# Autodesk Inventor assembly: GarageAndBracket
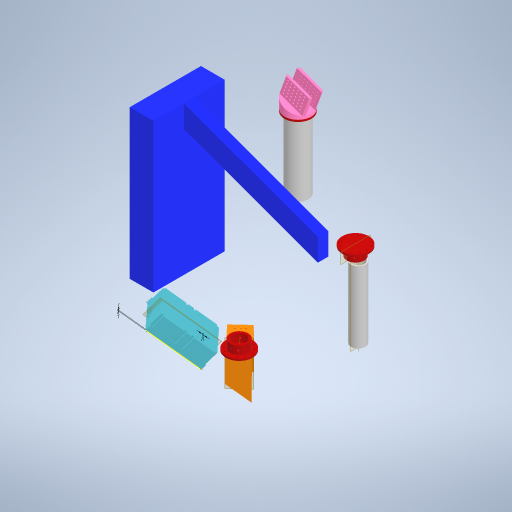
[picture p0: Inventor's stored thumbnail of the model, 512x512]
Saved by Autodesk Inventor 2023 (Build 270158030, 158C)
## iProperties
Created: 2021-11-26
Part Number: GarageAndBracket
Document SubType Name: Assembly
Designer: robst
Author: robst
## Documents named in this file (9)
- C:\git\CAD-Development\robSteele\ShapeWays\GlobalMeteorNetwork\GarageAndBracket.iam
- C:\git\CAD-Development\robSteele\ShapeWays\GlobalMeteorNetwork\GarageSegment.ipt
- C:\git\CAD-Development\robSteele\ShapeWays\GlobalMeteorNetwork\pvcBracketUpperPortionV02.ipt
- C:\git\CAD-Development\robSteele\ShapeWays\GlobalMeteorNetwork\topAttachementForPvcPipe.ipt
- C:\git\CAD-Development\robSteele\ShapeWays\GlobalMeteorNetwork\bracketForGarageLowerHalf.ipt
- C:\git\CAD-Development\robSteele\ShapeWays\GlobalMeteorNetwork\caseUpperPortion.ipt
- C:\git\CAD-Development\robSteele\ShapeWays\GlobalMeteorNetwork\3inchPvcPipe.ipt
- C:\git\CAD-Development\robSteele\ShapeWays\GlobalMeteorNetwork\2inchPvcForBracket.ipt
- C:\git\CAD-Development\robSteele\ShapeWays\GlobalMeteorNetwork\topAttachementFor2InchPvcPipe.ipt
## Components (9 placed, 8 different names)
1. GarageSegment:1 — Mate:13, Mate:14
2. 3inchPvcPipe:1 — Insert:2
3. topAttachementForPvcPipe:1 — Insert:2, Insert:3
4. topAttachementForPvcPipe:2 — Mate:11
5. bracketForGarageLowerHalf:1 — Mate:11, Mate:12, Flush:1
6. caseUpperPortion:1 — Mate:12, Flush:1
7. pvcBracketUpperPortionV02:1 — Mate:13, Mate:14, Insert:3
8. 2inchPvcForBracket:1
9. topAttachementFor2InchPvcPipe:1
## Relationships (7: Mate 4, Insert 2, Flush 1)
- Mate:11: topAttachementForPvcPipe:2 ↔ bracketForGarageLowerHalf:1
- Mate:12: bracketForGarageLowerHalf:1 ↔ caseUpperPortion:1
- Flush:1: bracketForGarageLowerHalf:1 ↔ caseUpperPortion:1
- Insert:2: 3inchPvcPipe:1 ↔ topAttachementForPvcPipe:1
- Mate:13: GarageSegment:1 ↔ pvcBracketUpperPortionV02:1
- Mate:14: GarageSegment:1 ↔ pvcBracketUpperPortionV02:1
- Insert:3: topAttachementForPvcPipe:1 ↔ pvcBracketUpperPortionV02:1
